# Autodesk Inventor assembly: MectoSYS_Rev1
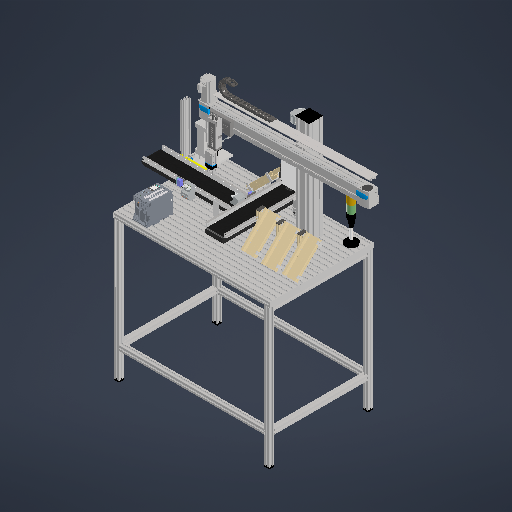
[picture p0: Inventor's stored thumbnail of the model, 512x512]
Saved by Autodesk Inventor 2027 (Build 310192000, 192)
## iProperties
Created: 2026-04-15
Part Number: MectoSYS_Rev1
Document SubType Name: Assembly
Designer: ratik
Author: ratik
## Documents named in this file (8)
- C:\Users\ratik\OneDrive\Personal Folder\00_Startup\00_MectoSYS_Repo\01_Mechanical_Design\01_CAD Design\3D file\Assembly File\MectoSYS_Rev1.iam
- C:\Users\ratik\OneDrive\Personal Folder\00_Startup\00_MectoSYS_Repo\01_Mechanical_Design\01_CAD Design\3D file\Assembly File\Base assembly.iam
- C:\Users\ratik\OneDrive\Personal Folder\00_Startup\00_MectoSYS_Repo\01_Mechanical_Design\01_CAD Design\3D file\Assembly File\Slider.iam
- C:\Users\ratik\OneDrive\Personal Folder\00_Startup\00_MectoSYS_Repo\01_Mechanical_Design\01_CAD Design\3D file\Assembly File\Conveyor Module.iam
- C:\Users\ratik\OneDrive\Personal Folder\00_Startup\00_MectoSYS_Repo\01_Mechanical_Design\01_CAD Design\3D file\Assembly File\Handlling Module.iam
- C:\Users\ratik\OneDrive\Personal Folder\00_Startup\00_MectoSYS_Repo\01_Mechanical_Design\01_CAD Design\3D file\Assembly File\Distribution module.iam
- C:\Users\ratik\OneDrive\Personal Folder\00_Startup\01_Mectosys_Prototype\01_Prototype\01_Mechanical\3D file\07_Comp\led-stack-light-indicator-signal-1.snapshot.3\Stack Light\Assembly Light Stack.iam
- C:\Users\ratik\Downloads\plc-s7-1500-model-6es7511-1ck00-0ab0-1.snapshot.1\6es75111ck000ab0\6es75111ck000ab0.ipt
## Components (11 placed, 7 different names)
1. Base assembly:1 [sub-assembly] — Mate:7, Mate:8, Mate:9, Mate:11, Mate:13, Mate:14, Mate:15, Mate:16
2. Conveyor Module:2 [sub-assembly] — Mate:8
3. Conveyor Module:3 [sub-assembly] — Mate:7
4. Handlling Module:1 [sub-assembly] — Mate:9, Mate:11
5. Slider:4 [sub-assembly] — Mate:13
6. Distribution module:1 [sub-assembly] — Mate:14
7. Assembly Light Stack:1 [sub-assembly] — Mate:15
8. 6es75111ck000ab0:1 — Mate:16
9. Slider:5 [sub-assembly]
10. Slider:6 [sub-assembly]
11. Slider:7 [sub-assembly]
## Relationships (8: Mate 8)
- Mate:7: Base assembly:1 ↔ Conveyor Module:3
- Mate:8: Base assembly:1 ↔ Conveyor Module:2
- Mate:9: Base assembly:1 ↔ Handlling Module:1
- Mate:11: Base assembly:1 ↔ Handlling Module:1
- Mate:13: Base assembly:1 ↔ Slider:4
- Mate:14: Base assembly:1 ↔ Distribution module:1
- Mate:15: Base assembly:1 ↔ Assembly Light Stack:1
- Mate:16: Base assembly:1 ↔ 6es75111ck000ab0:1
